# Autodesk Inventor assembly: top
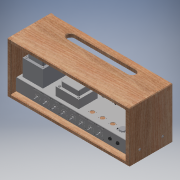
[picture p0: Inventor's stored thumbnail of the model, 180x180]
Saved by Autodesk Inventor 2016 (Build 200138000, 138)
## iProperties
Created: 2015-10-24
Part Number: top
Document SubType Name: Assembly
Designer: jeremyhale
Author: jeremyhale
## Documents named in this file (13)
- \\psf\Home\Documents\Poorhouse\git\p0001\top.iam
- \\psf\Home\Documents\Poorhouse\git\p0001\cabinet.iam
- \\psf\Home\Documents\Poorhouse\git\p0001\chassis.iam
- chassis.iam
- \\psf\Home\Documents\Poorhouse\git\p0001\cabinet-bottom.ipt
- \\psf\Home\Documents\Poorhouse\git\p0001\top\Design Accelerator\Bolted Connection7.iam
- \\psf\Home\Documents\Poorhouse\git\p0001\top\Design Accelerator\Bolted Connection8.iam
- \\psf\Home\Documents\Poorhouse\git\p0001\top\Design Accelerator\Bolted Connection9.iam
- \\psf\Home\Documents\Poorhouse\git\p0001\top\Design Accelerator\Bolted Connection12.iam
- \\psf\Home\Documents\Poorhouse\git\p0001\top\Design Accelerator\Bolted Connection13.iam
- \\psf\Home\Documents\Poorhouse\git\p0001\top\Design Accelerator\Bolted Connection15.iam
- \\psf\Home\Documents\Poorhouse\git\p0001\top\Design Accelerator\Bolted Connection14.iam
- \\psf\Home\Documents\Poorhouse\git\p0001\top\Design Accelerator\Bolted Connection16.iam
## Components (11 placed, 4 different names)
1. cabinet:1 [sub-assembly] — Flush:2, Flush:3, Flush:6, Flush:8, Flush:9, Mate:14, Mate:23, Mate:25, Mate:27, Mate:29
2. chassis:1 [sub-assembly] — Mate:1, Flush:4, Flush:5, Mate:16, Mate:18, Mate:20, Mate:22, Mate:24, Mate:26, Mate:28, Mate:30
3. cabinet-bottom:1 — Mate:1, Flush:4, Flush:5, Flush:6, Flush:8, Flush:9, Mate:14, Mate:15, Mate:17, Mate:19, Mate:21
4. Bolted Connection:1 [sub-assembly] — Mate:15, Mate:16
5. Bolted Connection:2 [sub-assembly] — Mate:17, Mate:18
6. Bolted Connection:3 [sub-assembly] — Mate:19, Mate:20
7. Bolted Connection:4 [sub-assembly] — Mate:21, Mate:22
8. Bolted Connection:5 [sub-assembly] — Mate:23, Mate:24
9. Bolted Connection:6 [sub-assembly] — Mate:25, Mate:26
10. Bolted Connection:7 [sub-assembly] — Mate:27, Mate:28
11. Bolted Connection:8 [sub-assembly] — Mate:29, Mate:30
## Relationships (25: Mate 18, Flush 7)
- Flush:2: cabinet:1
- Flush:3: cabinet:1
- Mate:1: chassis:1 ↔ cabinet-bottom:1
- Flush:4 (-25.4 mm): chassis:1 ↔ cabinet-bottom:1
- Flush:5: chassis:1 ↔ cabinet-bottom:1
- Flush:6: cabinet:1 ↔ cabinet-bottom:1
- Flush:8: cabinet:1 ↔ cabinet-bottom:1
- Flush:9: cabinet:1 ↔ cabinet-bottom:1
- Mate:14: cabinet:1 ↔ cabinet-bottom:1
- Mate:15: cabinet-bottom:1 ↔ Bolted Connection:1
- Mate:16: chassis:1 ↔ Bolted Connection:1
- Mate:17: cabinet-bottom:1 ↔ Bolted Connection:2
- Mate:18: chassis:1 ↔ Bolted Connection:2
- Mate:19: cabinet-bottom:1 ↔ Bolted Connection:3
- Mate:20: chassis:1 ↔ Bolted Connection:3
- Mate:21: cabinet-bottom:1 ↔ Bolted Connection:4
- Mate:22: chassis:1 ↔ Bolted Connection:4
- Mate:23: cabinet:1 ↔ Bolted Connection:5
- Mate:24: chassis:1 ↔ Bolted Connection:5
- Mate:25: cabinet:1 ↔ Bolted Connection:6
- Mate:26: chassis:1 ↔ Bolted Connection:6
- Mate:27: cabinet:1 ↔ Bolted Connection:7
- Mate:28: chassis:1 ↔ Bolted Connection:7
- Mate:29: cabinet:1 ↔ Bolted Connection:8
- Mate:30: chassis:1 ↔ Bolted Connection:8
